# Autodesk Inventor assembly: 151
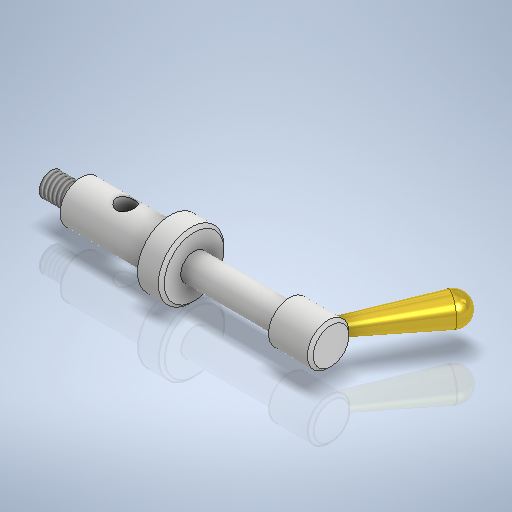
[picture p0: Inventor's stored thumbnail of the model, 512x512]
Saved by Autodesk Inventor 2025.1 (Build 291241000, 241)
## iProperties
Created: 2024-08-05
Part Number: 151
Document SubType Name: Assembly
Designer: ffogue
Author: ffogue
## Documents named in this file (3)
- C:\Projkete - Übungen\Freedom\151.iam
- C:\Projkete - Übungen\Freedom\151.ipt
- C:\Projkete - Übungen\Freedom\134 handle.ipt
## Components (2 placed, 2 different names)
1. 151:1 — Mate:1, Rotational:1
2. 134 handle:1 — Mate:1, Rotational:1
## Relationships (2: Mate 1, RevoluteJoint 1)
- Mate:1: 151:1 ↔ 134 handle:1
- Rotational:1 [RevoluteJoint] (-0.5 mm): 151:1 ↔ 134 handle:1
